# Autodesk Inventor assembly: Assembly
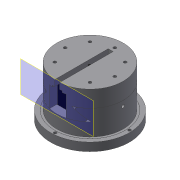
[picture p0: Inventor's stored thumbnail of the model, 180x180]
Saved by Autodesk Inventor 2018 (Build 220112000, 112)
## iProperties
Created: 2017-12-03
Part Number: Assembly
Document SubType Name: Assembly
Designer: Bardo91
Author: Bardo91
## Documents named in this file (5)
- E:\programming\hecatonquiros\cad_models\arm_3_dog\serial_model\Assembly.iam
- E:\programming\hecatonquiros\cad_models\arm_3_dog\serial_model\arm_0_attachment.ipt
- E:\programming\hecatonquiros\cad_models\arm_3_dog\serial_model\arm_0_top.ipt
- E:\programming\hecatonquiros\cad_models\arm_3_dog\serial_model\servo_FT_SC.ipt
- E:\programming\hecatonquiros\cad_models\arm_3_dog\serial_model\arm_0_bottom.ipt
## Components (4 placed, 4 different names)
1. arm_0_attachment:1 — Mate:1, Mate:2, Mate:3
2. arm_0_top:1 — Mate:1, Mate:2, Mate:3, Mate:4, Mate:5, Mate:6, Mate:7, Flush:1
3. servo_FT_SC:1 — Mate:4, Mate:5, Mate:6
4. arm_0_bottom:1 — Mate:7, Flush:1
## Relationships (8: Mate 7, Flush 1)
- Mate:1: arm_0_attachment:1 ↔ arm_0_top:1
- Mate:2: arm_0_attachment:1 ↔ arm_0_top:1
- Mate:3: arm_0_attachment:1 ↔ arm_0_top:1
- Mate:4: arm_0_top:1 ↔ servo_FT_SC:1
- Mate:5: arm_0_top:1 ↔ servo_FT_SC:1
- Mate:6: arm_0_top:1 ↔ servo_FT_SC:1
- Mate:7: arm_0_top:1 ↔ arm_0_bottom:1
- Flush:1: arm_0_top:1 ↔ arm_0_bottom:1
